# Autodesk Inventor assembly: motor_wheel_2
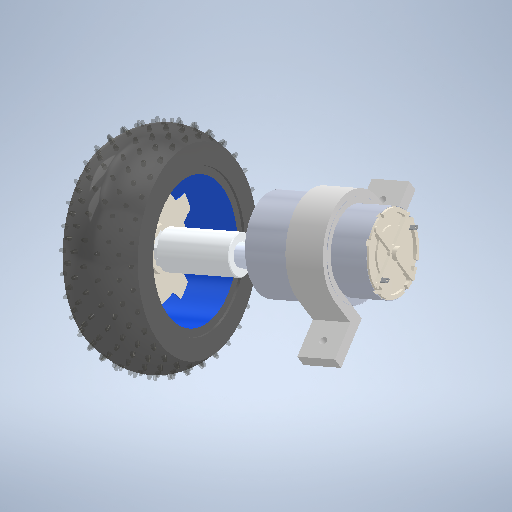
[picture p0: Inventor's stored thumbnail of the model, 512x512]
Saved by Autodesk Inventor 2025.3 (Build 293356030, 356C)
## iProperties
Created: 2026-06-28
Part Number: motor_wheel_2
Document SubType Name: Assembly
Designer: user
Author: user
## Documents named in this file (5)
- C:\Docs\shcool\dojo\Design_3\Smaller\motor_wheel_3.iam
- C:\Docs\shcool\dojo\Design_3\Smaller\U_BRACKET_2.ipt
- C:\Docs\shcool\dojo\Design_3\Smaller\gear motor.ipt
- C:\Docs\shcool\dojo\Design_3\Smaller\old_85mm_Wheel.ipt
- C:\Docs\shcool\dojo\Design_3\Smaller\Hub-12-Eixo6_aluminio.ipt
## Components (4 placed, 4 different names)
1. U_BRACKET_2:1 — Insert:2
2. gear motor:1 — Insert:1, Insert:2
3. old_85mm_Wheel:1 — Mate:1, Mate:2
4. Hub-12-Eixo6_aluminio:1 — Mate:1, Mate:2, Insert:1
## Relationships (4: Mate 2, Insert 2)
- Mate:1: old_85mm_Wheel:1 ↔ Hub-12-Eixo6_aluminio:1
- Mate:2: old_85mm_Wheel:1 ↔ Hub-12-Eixo6_aluminio:1
- Insert:1: gear motor:1 ↔ Hub-12-Eixo6_aluminio:1
- Insert:2: U_BRACKET_2:1 ↔ gear motor:1
